# Autodesk Inventor assembly: cnc_2mm_v1
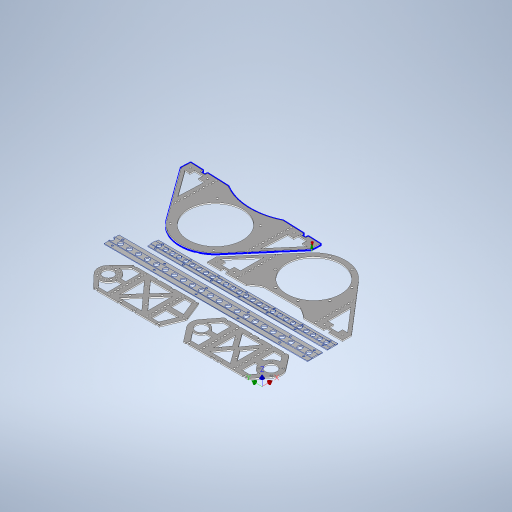
[picture p0: Inventor's stored thumbnail of the model, 512x512]
Saved by Autodesk Inventor 2024 (Build 280153000, 153)
## iProperties
Created: 2025-02-17
Part Number: cnc_2mm_v1
Document SubType Name: Assembly
Designer: tanoue_kota
Author: tanoue_kota
## Documents named in this file (7)
- C:\Users\田之上巧太\Documents\Inventor\RobArm\CNC\cnc_2mm_v1.iam
- C:\Users\田之上巧太\Documents\Inventor\RobArm\rob_link1\link1plate2.ipt
- C:\Users\田之上巧太\Documents\Inventor\RobArm\rob_link2\link2plate2.ipt
- C:\Users\田之上巧太\Documents\Inventor\RobArm\CNC\base_plate1\base_plate1.ipt
- C:\Users\田之上巧太\Documents\Inventor\RobArm\CNC\base_plate3\base_plate3.ipt
- C:\Users\田之上巧太\Documents\Inventor\RobArm\CNC\link1plate6\link1plate6.ipt
- C:\Users\田之上巧太\Documents\Inventor\RobArm\CNC\link2plate5\link2plate5.ipt
## Components (6 placed, 6 different names)
1. link1plate2:1 — フラッシュ:1, メイト:3, フラッシュ:5, フラッシュ:6, フラッシュ:7, メイト:4, メイト:5
2. link2plate2:1 — フラッシュ:1, フラッシュ:2, メイト:1, メイト:3, フラッシュ:4, フラッシュ:5
3. base_plate1:1 — フラッシュ:2, メイト:1, メイト:2, フラッシュ:3, フラッシュ:4
4. base_plate3:1 — メイト:2, フラッシュ:3
5. link1plate6:1 — フラッシュ:7, メイト:5
6. link2plate5:1 — フラッシュ:6, メイト:4
## Relationships (12: Flush 7, Mate 5)
- フラッシュ:1 [Flush]: link1plate2:1 ↔ link2plate2:1
- フラッシュ:2 [Flush]: link2plate2:1 ↔ base_plate1:1
- メイト:1 [Mate] (8 mm): link2plate2:1 ↔ base_plate1:1
- メイト:2 [Mate] (8 mm): base_plate1:1 ↔ base_plate3:1
- フラッシュ:3 [Flush]: base_plate1:1 ↔ base_plate3:1
- メイト:3 [Mate] (8 mm): link1plate2:1 ↔ link2plate2:1
- フラッシュ:4 [Flush]: link2plate2:1 ↔ base_plate1:1
- フラッシュ:5 [Flush]: link1plate2:1 ↔ link2plate2:1
- フラッシュ:6 [Flush]: link1plate2:1 ↔ link2plate5:1
- フラッシュ:7 [Flush]: link1plate2:1 ↔ link1plate6:1
- メイト:4 [Mate] (8 mm): link1plate2:1 ↔ link2plate5:1
- メイト:5 [Mate] (8 mm): link1plate2:1 ↔ link1plate6:1
